# Autodesk Inventor assembly: New_New_Spinning_Idea
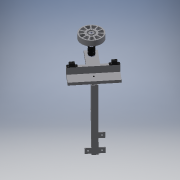
[picture p0: Inventor's stored thumbnail of the model, 180x180]
Saved by Autodesk Inventor 2017 (Build 210142000, 142)
## iProperties
Created: 2020-02-08
Part Number: New_New_Spinning_Idea
Document SubType Name: Assembly
Designer: S347110131
Author: S347110131
## Documents named in this file (7)
- \\ad.ocdsb.ca\studenthome\3\S338674153\FRC 2020\FullRobotRefactor\Control Panel\Panel_Spinning_Assembled.iam
- \\ad.ocdsb.ca\studenthome\3\S338674153\FRC 2020\FullRobotRefactor\Control Panel\2019-12-30+JE-PLG-149+with+adapter+R1.iam
- \\ad.ocdsb.ca\studenthome\3\S338674153\FRC 2020\FullRobotRefactor\Control Panel\NewNewMechanism.ipt
- \\ad.ocdsb.ca\studenthome\3\S338674153\FRC 2020\FullRobotRefactor\Control Panel\Color SensorREV-31-1557.iam
- \\ad.ocdsb.ca\studenthome\3\S338674153\FRC 2020\FullRobotRefactor\Control Panel\046-DP.iam
- \\ad.ocdsb.ca\studenthome\3\S338674153\FRC 2020\FullRobotRefactor\Control Panel\am-3480 4IN 500Hex Compliant Wheel REV2.iam
- \\ad.ocdsb.ca\studenthome\3\S338674153\FRC 2020\FullRobotRefactor\Control Panel\Mount for Control Panel.ipt
## Components (7 placed, 6 different names)
1. am-3480 4IN 500Hex Compliant Wheel REV2:1 [sub-assembly] — Mate:2, Mate:12
2. 2019-12-30+JE-PLG-149+with+adapter+R1:1 [sub-assembly] — Mate:1, Mate:2, Mate:12, Mate:17
3. NewNewMechanism:1 — Mate:1, Mate:5, Mate:7, Mate:8, Mate:9, Mate:10, Mate:11, Mate:14, Mate:15, Mate:17
4. Color SensorREV-31-1557:1 [sub-assembly] — Mate:7, Mate:8, Mate:15
5. Color SensorREV-31-1557:2 [sub-assembly] — Mate:5, Mate:11, Mate:14
6. 046-DP:1 [sub-assembly] — Mate:9, Mate:10, Mate:18, Mate:19
7. Mount for Control Panel:1 — Mate:18, Mate:19
## Relationships (14: Mate 14)
- Mate:1: 2019-12-30+JE-PLG-149+with+adapter+R1:1 ↔ NewNewMechanism:1
- Mate:2: am-3480 4IN 500Hex Compliant Wheel REV2:1 ↔ 2019-12-30+JE-PLG-149+with+adapter+R1:1
- Mate:5: NewNewMechanism:1 ↔ Color SensorREV-31-1557:2
- Mate:7: NewNewMechanism:1 ↔ Color SensorREV-31-1557:1
- Mate:8: NewNewMechanism:1 ↔ Color SensorREV-31-1557:1
- Mate:9: NewNewMechanism:1 ↔ 046-DP:1
- Mate:10: NewNewMechanism:1 ↔ 046-DP:1
- Mate:11: NewNewMechanism:1 ↔ Color SensorREV-31-1557:2
- Mate:12: am-3480 4IN 500Hex Compliant Wheel REV2:1 ↔ 2019-12-30+JE-PLG-149+with+adapter+R1:1
- Mate:14: NewNewMechanism:1 ↔ Color SensorREV-31-1557:2
- Mate:15: NewNewMechanism:1 ↔ Color SensorREV-31-1557:1
- Mate:17: 2019-12-30+JE-PLG-149+with+adapter+R1:1 ↔ NewNewMechanism:1
- Mate:18: 046-DP:1 ↔ Mount for Control Panel:1
- Mate:19 (3.81 mm): 046-DP:1 ↔ Mount for Control Panel:1
